# Autodesk Inventor assembly: SensorAssembly
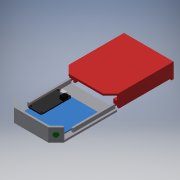
[picture p0: Inventor's stored thumbnail of the model, 180x180]
Saved by Autodesk Inventor 2018 (Build 220112000, 112)
## iProperties
Created: 2019-10-14
Part Number: SensorAssembly
Document SubType Name: Assembly
Designer: jklei
Author: jklei
## Documents named in this file (6)
- C:\Users\jklei\Desktop\Wildfire-Detector\CAD\SensorAssembly.iam
- C:\Users\jklei\Desktop\Wildfire-Detector\CAD\2829 Adafruit Feather Bluefruit 32u4.ipt
- C:\Users\jklei\Desktop\Wildfire-Detector\CAD\sensor.ipt
- C:\Users\jklei\Desktop\Wildfire-Detector\CAD\bottom-housing.ipt
- C:\Users\jklei\Desktop\Wildfire-Detector\CAD\top-slider.ipt
- C:\Users\jklei\Desktop\Wildfire-Detector\CAD\PCB.ipt
## Components (6 placed, 5 different names)
1. 2829 Adafruit Feather Bluefruit 32u4:1 — Flush:2, Flush:3, Mate:7
2. sensor:1 — Insert:2
3. sensor:2 — Insert:1
4. bottom-housing:1 — Flush:1, Mate:6, Insert:1, Insert:2, Mate:8, Mate:9, Mate:10
5. top-slider:1 — Flush:1, Mate:6
6. PCB:1 — Flush:2, Flush:3, Mate:7, Mate:8, Mate:9, Mate:10
## Relationships (10: Mate 5, Flush 3, Insert 2)
- Flush:1: bottom-housing:1 ↔ top-slider:1
- Mate:6: bottom-housing:1 ↔ top-slider:1
- Insert:1: sensor:2 ↔ bottom-housing:1
- Insert:2: sensor:1 ↔ bottom-housing:1
- Flush:2: 2829 Adafruit Feather Bluefruit 32u4:1 ↔ PCB:1
- Flush:3 (3.175 mm): 2829 Adafruit Feather Bluefruit 32u4:1 ↔ PCB:1
- Mate:7 (2.54 mm): 2829 Adafruit Feather Bluefruit 32u4:1 ↔ PCB:1
- Mate:8: bottom-housing:1 ↔ PCB:1
- Mate:9 (2.54 mm): bottom-housing:1 ↔ PCB:1
- Mate:10 (2.54 mm): bottom-housing:1 ↔ PCB:1
